# Autodesk Inventor assembly: 0.5 short version assembly
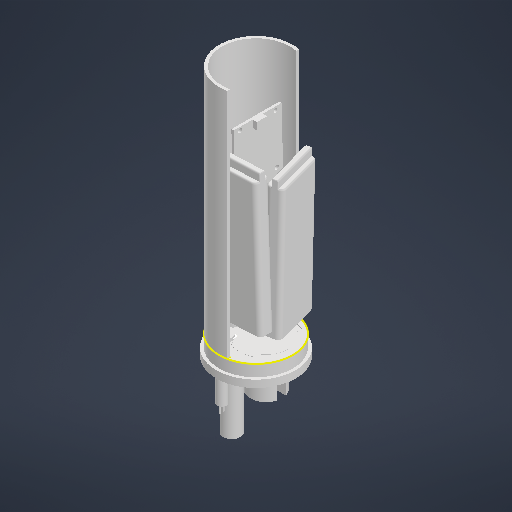
[picture p0: Inventor's stored thumbnail of the model, 512x512]
Saved by Autodesk Inventor 2026 (Build 300175050, 175E)
## iProperties
Created: 2025-08-07
Part Number: 0.5 short version assembly
Document SubType Name: Assembly
Designer: localuser
Author: localuser
## Documents named in this file (8)
- C:\Users\localuser\Documents\arts lab git\In-Situ-Water-Quality-Sensor\System_development\Jocassee\V0.5.1\Chassis\CAD model of Water Sensor\0.5 short version assembly.iam
- C:\Users\localuser\Documents\arts lab git\In-Situ-Water-Quality-Sensor\System_development\Jocassee\V0.5.1\Chassis\CAD model of Water Sensor\shortened chassis.ipt
- C:\Users\localuser\Documents\arts lab git\In-Situ-Water-Quality-Sensor\System_development\Jocassee\V0.5.1\Chassis\CAD model of Water Sensor\CADs for Water Sensor assembly\single cell battery.ipt
- C:\Users\localuser\Documents\arts lab git\In-Situ-Water-Quality-Sensor\System_development\Jocassee\V0.5.1\Chassis\CAD model of Water Sensor\CADs for Water Sensor assembly\PCB Board.ipt
- C:\Users\localuser\Documents\arts lab git\In-Situ-Water-Quality-Sensor\System_development\Jocassee\V0.5.1\Chassis\CAD model of Water Sensor\CADs for Water Sensor assembly\Temp Water Sensor.ipt
- C:\Users\localuser\Documents\arts lab git\In-Situ-Water-Quality-Sensor\System_development\Jocassee\V0.5.1\Chassis\CAD model of Water Sensor\CADs for Water Sensor assembly\Light Water Sensor.ipt
- C:\Users\localuser\Documents\arts lab git\In-Situ-Water-Quality-Sensor\System_development\Jocassee\V0.5.1\Chassis\CAD model of Water Sensor\CADs for Water Sensor assembly\Arc Water Sensor.ipt
- C:\Users\localuser\Documents\arts lab git\In-Situ-Water-Quality-Sensor\System_development\Jocassee\V0.5.1\Chassis\CAD model of Water Sensor\CADs for Water Sensor assembly\pH Sensor.ipt
## Components (8 placed, 7 different names)
1. shortened chassis:1 — Rigid:1, Rigid:2, Rigid:3, Rigid:4
2. single cell battery:1
3. single cell battery:2
4. PCB Board:1
5. Temp Water Sensor:1 — Rigid:3
6. Light Water Sensor:1 — Rigid:1
7. Arc Water Sensor:1 — Rigid:2
8. pH Sensor:1 — Rigid:4
## Relationships (4: WeldJoint 4)
- Rigid:1 [WeldJoint]: shortened chassis:1 ↔ Light Water Sensor:1
- Rigid:2 [WeldJoint] (2 mm): shortened chassis:1 ↔ Arc Water Sensor:1
- Rigid:3 [WeldJoint] (2 mm): shortened chassis:1 ↔ Temp Water Sensor:1
- Rigid:4 [WeldJoint] (54 mm): shortened chassis:1 ↔ pH Sensor:1
